# Autodesk Inventor assembly: N20Module
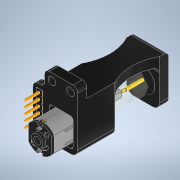
[picture p0: Inventor's stored thumbnail of the model, 180x180]
Saved by Autodesk Inventor 2022 (Build 260153000, 153)
## iProperties
Created: 2021-12-07
Part Number: N20Module
Document SubType Name: Assembly
Designer: JK
Author: JK
## Documents named in this file (6)
- C:\Users\FabLab\Desktop\JK\N20-Leg-Actuator\CADfiles\N20Module\N20Module.iam
- C:\Users\FabLab\Desktop\JK\N20-Leg-Actuator\CADfiles\N20Module\Case.ipt
- C:\Users\FabLab\Desktop\JK\N20-Leg-Actuator\CADfiles\N20Module\Brushed DC Motor v8.iam
- C:\Users\FabLab\Desktop\JK\N20-Leg-Actuator\CADfiles\N20Module\ServoPot.ipt
- C:\Users\FabLab\Desktop\JK\N20-Leg-Actuator\CADfiles\N20Module\Couple.ipt
- C:\Users\FabLab\Desktop\JK\N20-Leg-Actuator\CADfiles\N20Module\5pinheader.ipt
## Components (5 placed, 5 different names)
1. Case:1 — Coincidencia:1, Ángulo:1, Coincidencia:2, Coincidencia:6, Coincidencia:7, Nivelación:1
2. Brushed DC Motor v8:1 [sub-assembly] — Coincidencia:1, Ángulo:1, Coincidencia:2, Coincidencia:3, Coincidencia:5
3. ServoPot:1 — Coincidencia:3, Coincidencia:8
4. Couple:1 — Coincidencia:5, Coincidencia:8
5. 5pinheader:1 — Coincidencia:6, Coincidencia:7, Nivelación:1
## Relationships (9: Mate 7, Angle 1, Flush 1)
- Coincidencia:1 [Mate]: Case:1 ↔ Brushed DC Motor v8:1
- Ángulo:1 [Angle] (0 deg): Case:1 ↔ Brushed DC Motor v8:1
- Coincidencia:2 [Mate]: Case:1 ↔ Brushed DC Motor v8:1
- Coincidencia:3 [Mate]: Brushed DC Motor v8:1 ↔ ServoPot:1
- Coincidencia:5 [Mate]: Brushed DC Motor v8:1 ↔ Couple:1
- Coincidencia:6 [Mate] (0.1 mm): Case:1 ↔ 5pinheader:1
- Coincidencia:7 [Mate] (0.1 mm): Case:1 ↔ 5pinheader:1
- Nivelación:1 [Flush]: Case:1 ↔ 5pinheader:1
- Coincidencia:8 [Mate]: ServoPot:1 ↔ Couple:1
